# Autodesk Inventor assembly: Assembly OF STEVO MOTOR
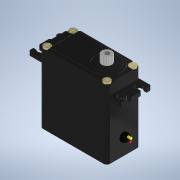
[picture p0: Inventor's stored thumbnail of the model, 180x180]
Saved by Autodesk Inventor 2022 (Build 260153000, 153)
## iProperties
Created: 2022-07-27
Part Number: Assembly OF STEVO MOTOR
Document SubType Name: Assembly
Designer: Dell
Author: Dell
## Documents named in this file (5)
- C:\Users\Dell\Documents\Assembly OF STEVO MOTOR.iam
- C:\Users\Dell\Documents\SERVO MOTOR PART1.ipt
- C:\Users\Dell\Documents\M3XT25.ipt
- C:\Users\Dell\Documents\SECROW SERVO.ipt
- C:\Users\Dell\Documents\servo wires.ipt
## Components (7 placed, 4 different names)
1. SERVO MOTOR PART1:1 — Rotational:1, Rigid:1, Insert:1, Insert:2, Insert:3, Rotational:2
2. M3XT25:1 — Rotational:1
3. SECROW SERVO:1 — Rigid:1
4. SECROW SERVO:2 — Insert:1
5. SECROW SERVO:3 — Insert:2
6. SECROW SERVO:4 — Insert:3
7. servo wires:1 — Rotational:2
## Relationships (6: Insert 3, RevoluteJoint 2, WeldJoint 1)
- Rotational:1 [RevoluteJoint]: SERVO MOTOR PART1:1 ↔ M3XT25:1
- Rigid:1 [WeldJoint]: SERVO MOTOR PART1:1 ↔ SECROW SERVO:1
- Insert:1: SERVO MOTOR PART1:1 ↔ SECROW SERVO:2
- Insert:2: SERVO MOTOR PART1:1 ↔ SECROW SERVO:3
- Insert:3: SERVO MOTOR PART1:1 ↔ SECROW SERVO:4
- Rotational:2 [RevoluteJoint]: SERVO MOTOR PART1:1 ↔ servo wires:1
